# Autodesk Inventor assembly: Assembly1
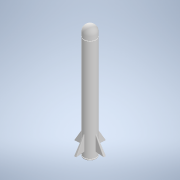
[picture p0: Inventor's stored thumbnail of the model, 180x180]
Saved by Autodesk Inventor 2022 (Build 260153000, 153)
## iProperties
Created: 2023-01-18
Part Number: Assembly1
Document SubType Name: Assembly
Designer: CLCK
Author: CLCK
## Documents named in this file (4)
- D:\Desktop\WorkSpace\torpedo-diy\CADs\final.iam
- D:\Desktop\WorkSpace\torpedo-diy\CADs\body.ipt
- D:\Desktop\WorkSpace\torpedo-diy\CADs\head.ipt
- D:\Desktop\WorkSpace\torpedo-diy\CADs\tale.ipt
## Components (3 placed, 3 different names)
1. body:1 — Insert:1, Insert:2
2. head:1 — Insert:1
3. tale:1 — Insert:2
## Relationships (2: Insert 2)
- Insert:1 (0.5 mm): body:1 ↔ head:1
- Insert:2 (0.5 mm): body:1 ↔ tale:1
